# Autodesk Inventor assembly: TorsoUnit
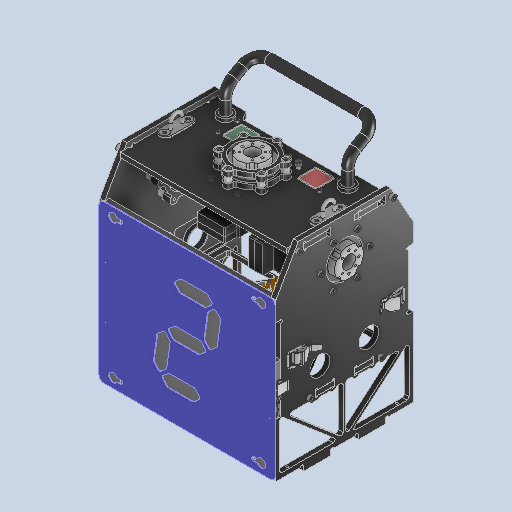
[picture p0: Inventor's stored thumbnail of the model, 512x512]
Saved by Autodesk Inventor 2024.2 (Build 282272000, 272)
## iProperties
Created: 2024-01-05
Part Number: TorsoUnit
Document SubType Name: Assembly
Designer: Masato Kubotera
Mass: 1439.76 g
Surface Area: 4091.65 cm^2
Volume: 567.798 cm^3
Density: 2.5357 g/cm^3
Author: Masato Kubotera
## Documents named in this file (22)
- C:\Users\masato\OneDrive - Chiba Institute of Technology\CIT Brains\RoboCup2024\Mechanic\SUSTAINA-OP2\NativeFiles\Boby\Torso\TorsoUnit.iam
- C:\Users\masato\OneDrive - Chiba Institute of Technology\CIT Brains\RoboCup2024\Mechanic\SUSTAINA-OP2\NativeFiles\Boby\CommonDesignedComponents\CrossRollerBearingUnit\CrossRollerBearingUnit.iam
- C:\Users\masato\OneDrive - Chiba Institute of Technology\CIT Brains\RoboCup2024\Mechanic\SUSTAINA-OP2\NativeFiles\Boby\COTS\Actuators\PMX-SCR-5204HV.ipt
- C:\Users\masato\OneDrive - Chiba Institute of Technology\CIT Brains\RoboCup2024\Mechanic\SUSTAINA-OP2\NativeFiles\Boby\Torso\TorsoUpperFrame.ipt
- C:\Users\masato\OneDrive - Chiba Institute of Technology\CIT Brains\RoboCup2024\Mechanic\SUSTAINA-OP2\NativeFiles\Boby\COTS\Washers\Metal\UZB.ipt
- C:\Users\masato\OneDrive - Chiba Institute of Technology\CIT Brains\RoboCup2024\Mechanic\SUSTAINA-OP2\NativeFiles\Boby\COTS\MisumiComponents\UHFNB125.ipt
- C:\Users\masato\OneDrive - Chiba Institute of Technology\CIT Brains\RoboCup2024\Mechanic\SUSTAINA-OP2\NativeFiles\Boby\COTS\Screws\CapScrew\UC-0515.ipt
- C:\Users\masato\OneDrive - Chiba Institute of Technology\CIT Brains\RoboCup2024\Mechanic\SUSTAINA-OP2\NativeFiles\Boby\COTS\Screws\CapScrew\FC-2615EB.ipt
- C:\Users\masato\OneDrive - Chiba Institute of Technology\CIT Brains\RoboCup2024\Mechanic\SUSTAINA-OP2\NativeFiles\Boby\Torso\TorsoFrontCoverFrame.ipt
- C:\Users\masato\OneDrive - Chiba Institute of Technology\CIT Brains\RoboCup2024\Mechanic\SUSTAINA-OP2\NativeFiles\Boby\Torso\TorsoColorMarker.ipt
- C:\Users\masato\OneDrive - Chiba Institute of Technology\CIT Brains\RoboCup2024\Mechanic\SUSTAINA-OP2\NativeFiles\Boby\Torso\TorsoLowerFrame.ipt
- C:\Users\masato\OneDrive - Chiba Institute of Technology\CIT Brains\RoboCup2024\Mechanic\SUSTAINA-OP2\NativeFiles\Boby\Torso\TorsoButtonCoverFrame.ipt
- C:\Users\masato\OneDrive - Chiba Institute of Technology\CIT Brains\RoboCup2024\Mechanic\SUSTAINA-OP2\NativeFiles\Boby\CustomElectronicComponents\SUSTAINA-BUTTON-MODULE.ipt
- C:\Users\masato\OneDrive - Chiba Institute of Technology\CIT Brains\RoboCup2024\Mechanic\SUSTAINA-OP2\NativeFiles\Boby\COTS\Screws\CapScrew\UC-0210.ipt
- C:\Users\masato\OneDrive - Chiba Institute of Technology\CIT Brains\RoboCup2024\Mechanic\SUSTAINA-OP2\NativeFiles\Boby\COTS\Screws\CapScrew\PCC-0306.ipt
- C:\Users\masato\OneDrive - Chiba Institute of Technology\CIT Brains\RoboCup2024\Mechanic\SUSTAINA-OP2\NativeFiles\Boby\COTS\MisumiComponents\TKC\TKC.ipt
- C:\Users\masato\OneDrive - Chiba Institute of Technology\CIT Brains\RoboCup2024\Mechanic\SUSTAINA-OP2\NativeFiles\Boby\COTS\ElectronicComponents\DK-42688-P\DK-42688-P.ipt
- C:\Users\masato\OneDrive - Chiba Institute of Technology\CIT Brains\RoboCup2024\Mechanic\SUSTAINA-OP2\NativeFiles\Boby\COTS\Bushes\D2030-5805B.ipt
- C:\Users\masato\OneDrive - Chiba Institute of Technology\CIT Brains\RoboCup2024\Mechanic\SUSTAINA-OP2\NativeFiles\Boby\COTS\Screws\CapScrew\UC-0204.ipt
- C:\Users\masato\OneDrive - Chiba Institute of Technology\CIT Brains\RoboCup2024\Mechanic\SUSTAINA-OP2\NativeFiles\Boby\Torso\TorsoSideUnit.iam
- C:\Users\masato\OneDrive - Chiba Institute of Technology\CIT Brains\RoboCup2024\Mechanic\SUSTAINA-OP2\NativeFiles\Boby\COTS\MisumiComponents\PKWS1_s.ipt
- C:\Users\masato\OneDrive - Chiba Institute of Technology\CIT Brains\RoboCup2024\Mechanic\SUSTAINA-OP2\NativeFiles\Boby\COTS\Screws\U-0205.ipt
## Components (42 placed, 21 different names)
1. CrossRollerBearingUnit:2 [sub-assembly] — Mate:1, Flush:3, Mate:2, Insert:152, Insert:153
2. TKC:1 — Insert:240, Insert:241
3. TKC:2 — Insert:242, Insert:243
4. DK-42688-P:1 — Mate:206, Mate:207, Mate:208
5. D2030-5805B:1 — Insert:244, Insert:248
6. D2030-5805B:2 — Insert:245, Insert:249
7. D2030-5805B:3 — Insert:246, Insert:250
8. D2030-5805B:4 — Insert:247, Insert:251
9. UC-0204:1 — Insert:248
10. UC-0204:2 — Insert:249
11. UC-0204:3 — Insert:250
12. UC-0204:4 — Insert:251
13. TorsoSideUnit:1 [sub-assembly] — Insert:254, Insert:255, Insert:258, Insert:259, Mate:209, Flush:5
14. TorsoSideUnit:2 [sub-assembly] — Insert:256, Insert:257, Insert:260, Insert:261, Flush:4
15. PKWS1_s:3 — Insert:289, Insert:290
16. U-0205:5
17. U-0205:6
18. PKWS1_s:4 — Insert:291, Insert:292
19. U-0205:7
20. U-0205:8
21. TorsoFrontCoverFrame:1 — Insert:285, Insert:286, Insert:287, Insert:288, Mate:209, Flush:4, Flush:5, Insert:289, Insert:290, Insert:291, Insert:292
22. TorsoColorMarker:1 — Insert:285, Insert:286, Insert:287, Insert:288
23. UHFNB125:1 — Insert:9, Insert:10
24. TorsoButtonCoverFrame:1 — Insert:208, Insert:209, Insert:210, Insert:211, Insert:212, Insert:213
25. TorsoUpperFrame:1 — Insert:152, Insert:153, Insert:154, Insert:155, Insert:156, Insert:157, Insert:158, Insert:159, Insert:160, Insert:161, Insert:210, Insert:211, Insert:212, Insert:213, Insert:214, Insert:215, Insert:216, Insert:217, Insert:218, Insert:219, Insert:220, Insert:221, Insert:240, Insert:241, Insert:242, Insert:243, Insert:254, Insert:255, Insert:256, Insert:257
26. TorsoLowerFrame:1 — Mate:206, Mate:207, Mate:208, Insert:244, Insert:245, Insert:246, Insert:247, Insert:258, Insert:259, Insert:260, Insert:261
27. SUSTAINA-BUTTON-MODULE:1 — Insert:208, Insert:209
28. PMX-SCR-5204HV:2 — Insert:154, Insert:155
29. UC-0210:1 — Insert:214
30. UC-0210:2 — Insert:215
31. UC-0210:3 — Insert:216
32. UC-0210:4 — Insert:217
33. UC-0515:1 — Insert:161
34. UC-0515:2 — Insert:160
35. FC-2615EB:3 — Insert:156
36. FC-2615EB:4 — Insert:157
37. PCC-0306:1 — Insert:218
38. PCC-0306:2 — Insert:219
39. PCC-0306:3 — Insert:220
40. PCC-0306:4 — Insert:221
41. UZB:1 — Insert:9, Insert:158
42. UZB:2 — Insert:10, Insert:159
## Relationships (67: Insert 58, Mate 6, Flush 3)
- Insert:9: UHFNB125:1 ↔ UZB:1
- Insert:10: UHFNB125:1 ↔ UZB:2
- Mate:1: CrossRollerBearingUnit:2
- Flush:3: CrossRollerBearingUnit:2
- Mate:2: CrossRollerBearingUnit:2
- Insert:152: CrossRollerBearingUnit:2 ↔ TorsoUpperFrame:1
- Insert:153: CrossRollerBearingUnit:2 ↔ TorsoUpperFrame:1
- Insert:154: TorsoUpperFrame:1 ↔ PMX-SCR-5204HV:2
- Insert:155: TorsoUpperFrame:1 ↔ PMX-SCR-5204HV:2
- Insert:156: TorsoUpperFrame:1 ↔ FC-2615EB:3
- Insert:157: TorsoUpperFrame:1 ↔ FC-2615EB:4
- Insert:158: TorsoUpperFrame:1 ↔ UZB:1
- Insert:159: TorsoUpperFrame:1 ↔ UZB:2
- Insert:160: TorsoUpperFrame:1 ↔ UC-0515:2
- Insert:161: TorsoUpperFrame:1 ↔ UC-0515:1
- Insert:208: TorsoButtonCoverFrame:1 ↔ SUSTAINA-BUTTON-MODULE:1
- Insert:209: TorsoButtonCoverFrame:1 ↔ SUSTAINA-BUTTON-MODULE:1
- Insert:210: TorsoButtonCoverFrame:1 ↔ TorsoUpperFrame:1
- Insert:211: TorsoButtonCoverFrame:1 ↔ TorsoUpperFrame:1
- Insert:212: TorsoButtonCoverFrame:1 ↔ TorsoUpperFrame:1
- Insert:213: TorsoButtonCoverFrame:1 ↔ TorsoUpperFrame:1
- Insert:214: TorsoUpperFrame:1 ↔ UC-0210:1
- Insert:215: TorsoUpperFrame:1 ↔ UC-0210:2
- Insert:216: TorsoUpperFrame:1 ↔ UC-0210:3
- Insert:217: TorsoUpperFrame:1 ↔ UC-0210:4
- Insert:218 (3 mm): TorsoUpperFrame:1 ↔ PCC-0306:1
- Insert:219 (3 mm): TorsoUpperFrame:1 ↔ PCC-0306:2
- Insert:220 (3 mm): TorsoUpperFrame:1 ↔ PCC-0306:3
- Insert:221 (3 mm): TorsoUpperFrame:1 ↔ PCC-0306:4
- Insert:240: TKC:1 ↔ TorsoUpperFrame:1
- Insert:241: TKC:1 ↔ TorsoUpperFrame:1
- Insert:242: TKC:2 ↔ TorsoUpperFrame:1
- Insert:243: TKC:2 ↔ TorsoUpperFrame:1
- Mate:206: DK-42688-P:1 ↔ TorsoLowerFrame:1
- Mate:207: DK-42688-P:1 ↔ TorsoLowerFrame:1
- Mate:208: DK-42688-P:1 ↔ TorsoLowerFrame:1
- Insert:244: D2030-5805B:1 ↔ TorsoLowerFrame:1
- Insert:245: D2030-5805B:2 ↔ TorsoLowerFrame:1
- Insert:246: D2030-5805B:3 ↔ TorsoLowerFrame:1
- Insert:247: D2030-5805B:4 ↔ TorsoLowerFrame:1
- Insert:248: D2030-5805B:1 ↔ UC-0204:1
- Insert:249: D2030-5805B:2 ↔ UC-0204:2
- Insert:250: D2030-5805B:3 ↔ UC-0204:3
- Insert:251: D2030-5805B:4 ↔ UC-0204:4
- Insert:254: TorsoSideUnit:1 ↔ TorsoUpperFrame:1
- Insert:255: TorsoSideUnit:1 ↔ TorsoUpperFrame:1
- Insert:256: TorsoSideUnit:2 ↔ TorsoUpperFrame:1
- Insert:257: TorsoSideUnit:2 ↔ TorsoUpperFrame:1
- Insert:258: TorsoSideUnit:1 ↔ TorsoLowerFrame:1
- Insert:259: TorsoSideUnit:1 ↔ TorsoLowerFrame:1
- Insert:260: TorsoSideUnit:2 ↔ TorsoLowerFrame:1
- Insert:261: TorsoSideUnit:2 ↔ TorsoLowerFrame:1
- [Insert]: PKWS1_s:3 ↔ U-0205:5
- [Insert]: PKWS1_s:3 ↔ U-0205:6
- [Insert]: PKWS1_s:4 ↔ U-0205:7
- [Insert]: PKWS1_s:4 ↔ U-0205:8
- Insert:285: TorsoFrontCoverFrame:1 ↔ TorsoColorMarker:1
- Insert:286: TorsoFrontCoverFrame:1 ↔ TorsoColorMarker:1
- Insert:287: TorsoFrontCoverFrame:1 ↔ TorsoColorMarker:1
- Insert:288: TorsoFrontCoverFrame:1 ↔ TorsoColorMarker:1
- Mate:209: TorsoSideUnit:1 ↔ TorsoFrontCoverFrame:1
- Flush:4: TorsoSideUnit:2 ↔ TorsoFrontCoverFrame:1
- Flush:5: TorsoSideUnit:1 ↔ TorsoFrontCoverFrame:1
- Insert:289: PKWS1_s:3 ↔ TorsoFrontCoverFrame:1
- Insert:290: PKWS1_s:3 ↔ TorsoFrontCoverFrame:1
- Insert:291: PKWS1_s:4 ↔ TorsoFrontCoverFrame:1
- Insert:292: PKWS1_s:4 ↔ TorsoFrontCoverFrame:1
## Named parameters: d341_d132 = 0 mm, d342_d133 = 0 mm, d343_d332_d132 = 0 mm, d344_d333_d133 = 0 mm
